# Autodesk Inventor assembly: Arm Segments Positioning Assembly
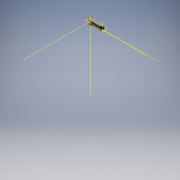
[picture p0: Inventor's stored thumbnail of the model, 180x180]
Saved by Autodesk Inventor 2019 (Build 230136000, 136)
## iProperties
Created: 2021-05-09
Part Number: Arm Segments Positioning Assembly
Document SubType Name: Assembly
Designer: Eric
Author: Eric
## Documents named in this file (8)
- C:\Users\Eric\Documents\! - Uni\Year 4\MENG-Robot-Fab-Project\Denavit-Hartneberg Tests\Models\ArmSegments\Arm Segments Positioning Assembly.iam
- C:\Users\Eric\Documents\! - Uni\Year 4\MENG-Robot-Fab-Project\Denavit-Hartneberg Tests\Models\ArmSegments\UR5_link_1.ipt
- C:\Users\Eric\Documents\! - Uni\Year 4\MENG-Robot-Fab-Project\Denavit-Hartneberg Tests\Models\ArmSegments\UR5_link_2.ipt
- C:\Users\Eric\Documents\! - Uni\Year 4\MENG-Robot-Fab-Project\Denavit-Hartneberg Tests\Models\ArmSegments\UR5_link_3.ipt
- C:\Users\Eric\Documents\! - Uni\Year 4\MENG-Robot-Fab-Project\Denavit-Hartneberg Tests\Models\ArmSegments\UR5_link_4.ipt
- C:\Users\Eric\Documents\! - Uni\Year 4\MENG-Robot-Fab-Project\Denavit-Hartneberg Tests\Models\ArmSegments\UR5_link_5.ipt
- C:\Users\Eric\Documents\! - Uni\Year 4\MENG-Robot-Fab-Project\Denavit-Hartneberg Tests\Models\ArmSegments\UR5_link_6.ipt
- C:\Users\Eric\Documents\! - Uni\Year 4\MENG-Robot-Fab-Project\Denavit-Hartneberg Tests\Models\ArmSegments\Space Envelope 1mm Aperture.ipt
## Components (7 placed, 7 different names)
1. Space Envelope 1mm Aperture:1 — Mate:11, Mate:12, Mate:13, Angle:4
2. UR5_link_1:1 — Mate:1, Mate:2, Angle:1
3. UR5_link_2:1 — Mate:3, Angle:2, Flush:1
4. UR5_link_3:1 — Angle:3, Mate:14, Mate:15
5. UR5_link_4:1 — Mate:7, Mate:6
6. UR5_link_5:1 — Mate:8, Mate:9
7. UR5_link_6:1 — Mate:10, Mate:11, Mate:12
## Relationships (18: Mate 13, Angle 4, Flush 1)
- Mate:1: UR5_link_1:1
- Mate:2: UR5_link_1:1
- Angle:1 (180 deg): UR5_link_1:1
- Mate:3: UR5_link_2:1
- Angle:2 (180 deg): UR5_link_2:1
- Flush:1: UR5_link_2:1
- Angle:3 (180 deg): UR5_link_3:1
- Mate:7: UR5_link_4:1
- Mate:6: UR5_link_4:1
- Mate:8: UR5_link_5:1
- Mate:9: UR5_link_5:1
- Mate:10: UR5_link_6:1
- Mate:11: Space Envelope 1mm Aperture:1 ↔ UR5_link_6:1
- Mate:12: Space Envelope 1mm Aperture:1 ↔ UR5_link_6:1
- Mate:13: Space Envelope 1mm Aperture:1
- Angle:4 (180 deg): Space Envelope 1mm Aperture:1
- Mate:14: UR5_link_3:1
- Mate:15: UR5_link_3:1
